# Autodesk Inventor assembly: Assembly1
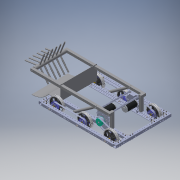
[picture p0: Inventor's stored thumbnail of the model, 180x180]
Saved by Autodesk Inventor 2016 (Build 200138000, 138)
## iProperties
Created: 2016-09-04
Part Number: Assembly1
Document SubType Name: Assembly
Designer: gus
Author: gus
## Documents named in this file (13)
- \\Mac\Home\Desktop\bunnybots 2016\prototype\Assembly1.iam
- \\Mac\Home\Desktop\bunnybots 2016\prototype\C-Base2LongTBMini6HiGripBelts.iam
- \\Mac\Home\Desktop\bunnybots 2016\prototype\Part88.ipt
- \\Mac\Home\Desktop\bunnybots 2016\prototype\Part89.ipt
- \\Mac\Home\Desktop\bunnybots 2016\prototype\Part88_MIR.ipt
- \\Mac\Home\Desktop\bunnybots 2016\prototype\Part89_MIR.ipt
- \\Mac\Home\Desktop\bunnybots 2016\prototype\Part93.ipt
- \\Mac\Home\Desktop\bunnybots 2016\prototype\Part95.ipt
- \\Mac\Home\Desktop\bunnybots 2016\prototype\Part1.ipt
- \\Mac\Home\Desktop\bunnybots 2016\prototype\Part2.ipt
- \\Mac\Home\Desktop\bunnybots 2016\prototype\Part1_MIR.ipt
- \\Mac\Home\Desktop\bunnybots 2016\prototype\Part2_MIR.ipt
- \\Mac\Home\Desktop\bunnybots 2016\prototype\Part4.ipt
## Components (29 placed, 12 different names)
1. C-Base2LongTBMini6HiGripBelts:1 [sub-assembly] — Flush:4, Mate:2, Mate:3, Mate:5, Flush:7, Flush:8, Mate:8, Tangent:2, Mate:13, Tangent:3, Mate:14
2. Part88:2 — Flush:4, Mate:2, Flush:5, Cylindrical:1, Mate:3, Mate:5, Flush:9
3. Part89:1 — Flush:5, Cylindrical:1, Cylindrical:10, Mate:16
4. Part88_MIR:1 — Mate:7, Cylindrical:2, Flush:8, Flush:9, Mate:8
5. Part89_MIR:1 — Mate:7, Cylindrical:2, Flush:10, Cylindrical:3, Cylindrical:7, Flush:11, Mate:16, Angle:1
6. Part93:1 — Flush:10, Cylindrical:3, Mate:10, Mate:11, Tangent:1, Mate:15
7. Part1:1 — Cylindrical:4, Tangent:2, Mate:13
8. Part2:1 — Cylindrical:4, Cylindrical:7
9. Part1_MIR:1 — Cylindrical:8, Tangent:3, Mate:14
10. Part2_MIR:1 — Cylindrical:8, Cylindrical:10
11. Part4:1 — Flush:11, Mate:15, Angle:1
12. Part95:1 — Mate:10, Mate:11, Tangent:1
13. Part95:2
14. Part95:3
15. Part95:4
16. Part95:5
17. Part95:6
18. Part95:7
19. Part95:8
20. Part95:9
21. Part95:10
22. Part95:11
23. Part95:12
24. Part95:13
25. Part95:14
26. Part95:15
27. Part95:16
28. Part95:17
29. Part95:18
## Component patterns: (3 elements), (6 elements, first: Part95:1), Component Pattern 1:2 (6 elements), Component Pattern 1:3 (6 elements)
## Relationships (29: Mate 11, Flush 7, CylindricalJoint 7, Tangent 3, Angle 1)
- Flush:4: C-Base2LongTBMini6HiGripBelts:1 ↔ Part88:2
- Mate:2: C-Base2LongTBMini6HiGripBelts:1 ↔ Part88:2
- Flush:5: Part88:2 ↔ Part89:1
- Cylindrical:1: Part88:2 ↔ Part89:1
- Mate:3: C-Base2LongTBMini6HiGripBelts:1 ↔ Part88:2
- Mate:5: C-Base2LongTBMini6HiGripBelts:1 ↔ Part88:2
- Flush:7 (-292.1 mm): C-Base2LongTBMini6HiGripBelts:1
- Mate:7: Part88_MIR:1 ↔ Part89_MIR:1
- Cylindrical:2: Part88_MIR:1 ↔ Part89_MIR:1
- Flush:8: C-Base2LongTBMini6HiGripBelts:1 ↔ Part88_MIR:1
- Flush:9: Part88:2 ↔ Part88_MIR:1
- Mate:8: C-Base2LongTBMini6HiGripBelts:1 ↔ Part88_MIR:1
- Flush:10: Part89_MIR:1 ↔ Part93:1
- Cylindrical:3: Part89_MIR:1 ↔ Part93:1
- Mate:10: Part93:1 ↔ Part95:1
- Mate:11: Part93:1 ↔ Part95:1
- Tangent:1 (50.8 mm): Part93:1 ↔ Part95:1
- Cylindrical:4: Part1:1 ↔ Part2:1
- Tangent:2: C-Base2LongTBMini6HiGripBelts:1 ↔ Part1:1
- Cylindrical:7: Part89_MIR:1 ↔ Part2:1
- Cylindrical:8: Part1_MIR:1 ↔ Part2_MIR:1
- Cylindrical:10: Part89:1 ↔ Part2_MIR:1
- Mate:13: C-Base2LongTBMini6HiGripBelts:1 ↔ Part1:1
- Tangent:3: C-Base2LongTBMini6HiGripBelts:1 ↔ Part1_MIR:1
- Mate:14: C-Base2LongTBMini6HiGripBelts:1 ↔ Part1_MIR:1
- Flush:11: Part89_MIR:1 ↔ Part4:1
- Mate:15: Part93:1 ↔ Part4:1
- Mate:16: Part89:1 ↔ Part89_MIR:1
- Angle:1 (90 deg): Part89_MIR:1 ↔ Part4:1
